# Autodesk Inventor assembly: Body Cap Subassembly
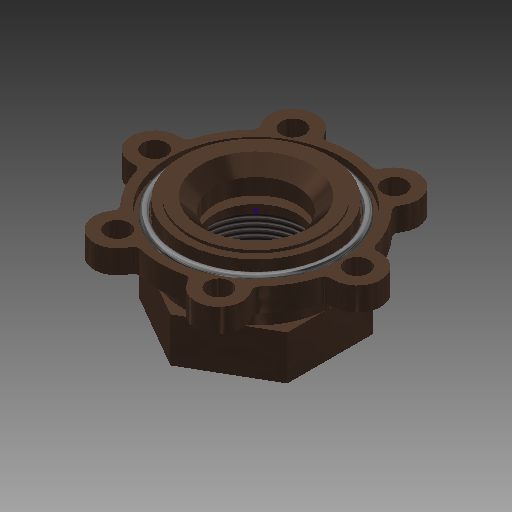
[picture p0: Inventor's stored thumbnail of the model, 512x512]
Saved by Autodesk Inventor 2018 (Build 220112000, 112)
## iProperties
Created: 2017-10-19
Part Number: Body Cap Subassembly
Document SubType Name: Assembly
Designer: kurtis
Author: kurtis
## Documents named in this file (5)
- D:\Users\kurti\Git-Home\CAD\GE101\MA9\Body Cap Subassembly.iam
- D:\Users\kurti\Git-Home\CAD\GE101\MA9\Seat.ipt
- D:\Users\kurti\Git-Home\CAD\GE101\MA9\Body Cap.ipt
- D:\Users\kurti\Git-Home\CAD\GE101\MA9\Oring1.ipt
- D:\Users\kurti\Git-Home\CAD\GE101\MA9\Spring.ipt
## Components (4 placed, 4 different names)
1. Seat:1 — Rigid:2, Rotational:1
2. Body Cap:1 — Rigid:1, Rigid:2
3. Oring1:1 — Rigid:1
4. Spring:1 — Rotational:1
## Relationships (3: WeldJoint 2, RevoluteJoint 1)
- Rigid:1 [WeldJoint] (1.5 mm): Body Cap:1 ↔ Oring1:1
- Rigid:2 [WeldJoint]: Seat:1 ↔ Body Cap:1
- Rotational:1 [RevoluteJoint]: Seat:1 ↔ Spring:1
